# Autodesk Inventor assembly: Assembly_Cube_empty_1x1_v2
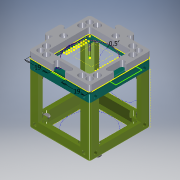
[picture p0: Inventor's stored thumbnail of the model, 180x180]
Saved by Autodesk Inventor 2019 (Build 230136000, 136)
## iProperties
Created: 2018-06-11
Part Number: Assembly_Cube_empty_1x1_v2
Material: Generisch
Document SubType Name: Assembly
Designer: diederichbenedict
Mass: 28.3962 g
Surface Area: 161.576 cm^2
Volume: 24.38 cm^3
Density: 1.16473 g/cm^3
Author: diederichbenedict
## Documents named in this file (7)
- C:\Users\UC2\Dropbox\UC2\02_CAD\INVENTOR\uc2_v3\Assembly_Cube_empty_1x1_withBase_v3.iam
- C:\Users\UC2\Dropbox\UC2\02_CAD\INVENTOR\uc2_v3\10_Cube_1x1_v3.ipt
- C:\Users\UC2\Dropbox\UC2\02_CAD\INVENTOR\uc2_v3\10_Lid_1x1_v3.ipt
- C:\Users\UC2\Dropbox\UC2\02_CAD\INVENTOR\uc2_v3\openSIMv3\BAK\DIN 912 - M3 x 0,5 x 12 x 10,75.ipt
- C:\Users\UC2\Documents\Inventor\Content Center Files\R2019\de-DE\ISO 4026\ISO 4026 - M5 x 8 - ISO.ipt
- C:\Users\UC2\Documents\Inventor\Content Center Files\R2019\de-DE\DIN 912\DIN 912 - M3 x 0,5 x 8 x 6,75.ipt
- C:\Users\UC2\Dropbox\UC2\02_CAD\INVENTOR\uc2_v3\10_Base_puzzle_v3.ipt
## Components (17 placed, 6 different names)
1. 10_Cube_1x1_v3:1 — Mate:3, Mate:2, Angle:3, Mate:4, Mate:5, Mate:6, Mate:7, Flush:9, Mate:8, Mate:9, Mate:10, Flush:12
2. 10_Lid_1x1_v3:1 — Mate:3, Mate:2, Flush:3, Flush:4, Flush:5, Insert:20, Insert:21, Insert:22, Insert:23, Angle:3, Mate:11, Mate:12, Mate:13, Flush:15, Mate:14, Angle:4, Mate:15
3. DIN 912 - ersetzt durch DIN EN ISO 4762 M3 x 12:5 — Insert:21
4. DIN 912 - ersetzt durch DIN EN ISO 4762 M3 x 12:6 — Insert:23
5. DIN 912 - ersetzt durch DIN EN ISO 4762 M3 x 12:7 — Insert:20
6. DIN 912 - ersetzt durch DIN EN ISO 4762 M3 x 12:8 — Insert:22
7. ISO 4026 M5 x 8:1 — Mate:8, Flush:10, Flush:11, Flush:12
8. ISO 4026 M5 x 8:2 — Mate:9, Flush:10
9. ISO 4026 M5 x 8:3 — Mate:10, Flush:11
10. ISO 4026 M5 x 8:4 — Mate:13, Flush:13
11. ISO 4026 M5 x 8:5 — Mate:11, Flush:14
12. ISO 4026 M5 x 8:6 — Mate:12, Flush:13, Flush:14, Flush:15
13. DIN 912 - ersetzt durch DIN EN ISO 4762 M3 x 8:1 — Mate:4, Flush:6, Flush:7, Flush:8, Flush:9
14. DIN 912 - ersetzt durch DIN EN ISO 4762 M3 x 8:2 — Mate:5, Flush:7
15. DIN 912 - ersetzt durch DIN EN ISO 4762 M3 x 8:3 — Mate:6, Flush:6
16. DIN 912 - ersetzt durch DIN EN ISO 4762 M3 x 8:4 — Mate:7, Flush:8
17. 10_Base_puzzle_v3:1 — Mate:14, Angle:4, Mate:15
## Relationships (33: Mate 14, Flush 13, Insert 4, Angle 2)
- Mate:3: 10_Cube_1x1_v3:1 ↔ 10_Lid_1x1_v3:1
- Mate:2: 10_Cube_1x1_v3:1 ↔ 10_Lid_1x1_v3:1
- Flush:3: 10_Lid_1x1_v3:1
- Flush:4: 10_Lid_1x1_v3:1
- Flush:5: 10_Lid_1x1_v3:1
- Insert:20: 10_Lid_1x1_v3:1 ↔ DIN 912 - ersetzt durch DIN EN ISO 4762 M3 x 12:7
- Insert:21: 10_Lid_1x1_v3:1 ↔ DIN 912 - ersetzt durch DIN EN ISO 4762 M3 x 12:5
- Insert:22: 10_Lid_1x1_v3:1 ↔ DIN 912 - ersetzt durch DIN EN ISO 4762 M3 x 12:8
- Insert:23: 10_Lid_1x1_v3:1 ↔ DIN 912 - ersetzt durch DIN EN ISO 4762 M3 x 12:6
- Angle:3 (0 deg): 10_Cube_1x1_v3:1 ↔ 10_Lid_1x1_v3:1
- Mate:4: 10_Cube_1x1_v3:1 ↔ DIN 912 - ersetzt durch DIN EN ISO 4762 M3 x 8:1
- Mate:5: 10_Cube_1x1_v3:1 ↔ DIN 912 - ersetzt durch DIN EN ISO 4762 M3 x 8:2
- Mate:6: 10_Cube_1x1_v3:1 ↔ DIN 912 - ersetzt durch DIN EN ISO 4762 M3 x 8:3
- Mate:7: 10_Cube_1x1_v3:1 ↔ DIN 912 - ersetzt durch DIN EN ISO 4762 M3 x 8:4
- Flush:6: DIN 912 - ersetzt durch DIN EN ISO 4762 M3 x 8:1 ↔ DIN 912 - ersetzt durch DIN EN ISO 4762 M3 x 8:3
- Flush:7: DIN 912 - ersetzt durch DIN EN ISO 4762 M3 x 8:1 ↔ DIN 912 - ersetzt durch DIN EN ISO 4762 M3 x 8:2
- Flush:8: DIN 912 - ersetzt durch DIN EN ISO 4762 M3 x 8:1 ↔ DIN 912 - ersetzt durch DIN EN ISO 4762 M3 x 8:4
- Flush:9: 10_Cube_1x1_v3:1 ↔ DIN 912 - ersetzt durch DIN EN ISO 4762 M3 x 8:1
- Mate:8: 10_Cube_1x1_v3:1 ↔ ISO 4026 M5 x 8:1
- Mate:9: 10_Cube_1x1_v3:1 ↔ ISO 4026 M5 x 8:2
- Mate:10: 10_Cube_1x1_v3:1 ↔ ISO 4026 M5 x 8:3
- Flush:10: ISO 4026 M5 x 8:1 ↔ ISO 4026 M5 x 8:2
- Flush:11: ISO 4026 M5 x 8:1 ↔ ISO 4026 M5 x 8:3
- Flush:12 (-2 mm): 10_Cube_1x1_v3:1 ↔ ISO 4026 M5 x 8:1
- Mate:11: 10_Lid_1x1_v3:1 ↔ ISO 4026 M5 x 8:5
- Mate:12: 10_Lid_1x1_v3:1 ↔ ISO 4026 M5 x 8:6
- Mate:13: 10_Lid_1x1_v3:1 ↔ ISO 4026 M5 x 8:4
- Flush:13: ISO 4026 M5 x 8:4 ↔ ISO 4026 M5 x 8:6
- Flush:14: ISO 4026 M5 x 8:5 ↔ ISO 4026 M5 x 8:6
- Flush:15 (-2 mm): 10_Lid_1x1_v3:1 ↔ ISO 4026 M5 x 8:6
- Mate:14: 10_Lid_1x1_v3:1 ↔ 10_Base_puzzle_v3:1
- Angle:4 (0 deg): 10_Lid_1x1_v3:1 ↔ 10_Base_puzzle_v3:1
- Mate:15: 10_Lid_1x1_v3:1 ↔ 10_Base_puzzle_v3:1
